# Autodesk Inventor assembly: Сборка1
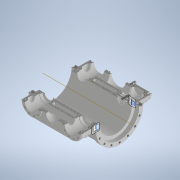
[picture p0: Inventor's stored thumbnail of the model, 180x180]
Saved by Autodesk Inventor 2021 (Build 250183000, 183)
## iProperties
Created: 2020-11-15
Part Number: Сборка1
Document SubType Name: Assembly
Designer: Тимоха
Author: Тимоха
## Documents named in this file (11)
- C:\Users\Тимоха\Desktop\КР Компрессор\МОЕ\Сборка1.iam
- C:\Users\Тимоха\Desktop\КР Компрессор\МОЕ\Цилиндр2.ipt
- C:\Users\Тимоха\Desktop\КР Компрессор\МОЕ\Прокладка рубашки охлаждения.ipt
- C:\Users\Тимоха\Desktop\КР Компрессор\МОЕ\Крышка рубашки охлаждения.ipt
- C:\Users\Тимоха\Documents\Inventor\Content Center Files\R2021\ru-RU\Bolt GOST R 50274-92\Болт M8-6g×20-F ГОСТ Р 50274-92.ipt
- C:\Users\Тимоха\Desktop\КР Компрессор\МОЕ\Клапан2.iam
- C:\Users\Тимоха\Desktop\КР Компрессор\МОЕ\Стакан1.ipt
- C:\Users\Тимоха\Desktop\КР Компрессор\МОЕ\Крышка стакана.ipt
- C:\Users\Тимоха\Documents\Inventor\Content Center Files\R2021\ru-RU\Stud GOST 22034-76\Шпилька M20-6g×50 ГОСТ 22034-76.ipt
- C:\Users\Тимоха\Documents\Inventor\Content Center Files\R2021\ru-RU\GOST 10450-78\Шайба 21 ГОСТ 10450-78.ipt
- C:\Users\Тимоха\Documents\Inventor\Content Center Files\R2021\ru-RU\GOST 15521-70\Гайка M20-6H ГОСТ 15521-70.ipt
## Components (11 placed, 10 different names)
1. Цилиндр2:1 — Заподлицо:1, Заподлицо:2, Жесткий:1, Жесткий:2, Жесткий:3, С поворотом:1, Цилиндрический:1
2. Прокладка рубашки охлаждения:1 — Заподлицо:2, Заподлицо:3, Жесткий:2, Заподлицо:4, Заподлицо:5
3. Прокладка рубашки охлаждения:2 — Жесткий:1
4. Крышка рубашки охлаждения:1 — Заподлицо:4, Заподлицо:5
5. Болт ГОСТ Р 50274-92 M8-6g×20-F:1 — Жесткий:3
6. Клапан2:1 [sub-assembly] — С поворотом:1, Жесткий:4
7. Стакан1:1 — Жесткий:4, С поворотом:2
8. Крышка стакана:1 — С поворотом:2, С поворотом:3
9. Шпилька ГОСТ 22034-76 M20-6g×50:1 — Цилиндрический:1
10. Шайба ГОСТ 10450-78 21:1 — С поворотом:3, С поворотом:4
11. Гайка ГОСТ 15521-70 M20:1 — С поворотом:4
## Relationships (14: Flush 5, WeldJoint 4, RevoluteJoint 4, CylindricalJoint 1)
- Заподлицо:1 [Flush] (150.75 mm): Цилиндр2:1
- Заподлицо:2 [Flush]: Цилиндр2:1 ↔ Прокладка рубашки охлаждения:1
- Заподлицо:3 [Flush]: Прокладка рубашки охлаждения:1
- Жесткий:1 [WeldJoint]: Цилиндр2:1 ↔ Прокладка рубашки охлаждения:2
- Жесткий:2 [WeldJoint]: Цилиндр2:1 ↔ Прокладка рубашки охлаждения:1
- Заподлицо:4 [Flush]: Прокладка рубашки охлаждения:1 ↔ Крышка рубашки охлаждения:1
- Заподлицо:5 [Flush]: Прокладка рубашки охлаждения:1 ↔ Крышка рубашки охлаждения:1
- Жесткий:3 [WeldJoint] (5 mm): Цилиндр2:1 ↔ Болт ГОСТ Р 50274-92 M8-6g×20-F:1
- С поворотом:1 [RevoluteJoint]: Цилиндр2:1 ↔ Клапан2:1
- Жесткий:4 [WeldJoint]: Клапан2:1 ↔ Стакан1:1
- С поворотом:2 [RevoluteJoint]: Стакан1:1 ↔ Крышка стакана:1
- Цилиндрический:1 [CylindricalJoint]: Цилиндр2:1 ↔ Шпилька ГОСТ 22034-76 M20-6g×50:1
- С поворотом:3 [RevoluteJoint]: Крышка стакана:1 ↔ Шайба ГОСТ 10450-78 21:1
- С поворотом:4 [RevoluteJoint]: Шайба ГОСТ 10450-78 21:1 ↔ Гайка ГОСТ 15521-70 M20:1
